# Autodesk Inventor assembly: black-suspension_MIR
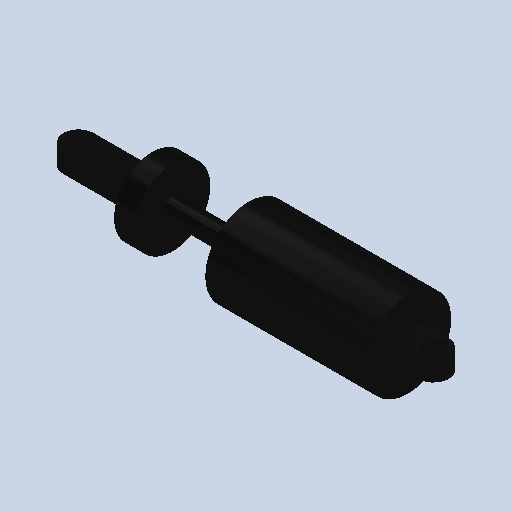
[picture p0: Inventor's stored thumbnail of the model, 512x512]
Saved by Autodesk Inventor 2025.1 (Build 291241000, 241)
## iProperties
Created: 2023-11-21
Part Number: black-suspension_MIR
Document SubType Name: Assembly
Designer: haruy
Author: haruy
## Documents named in this file (3)
- C:\Users\haruy\Documents\ロボコン\NHK2025\cad\000_parts\サスペンション\black-suspension_MIR.iam
- C:\Users\haruy\Documents\ロボコン\NHK2025\cad\000_parts\サスペンション\black-suspension-top_MIR.ipt
- C:\Users\haruy\Documents\ロボコン\NHK2025\cad\000_parts\サスペンション\black-suspension-under_MIR.ipt
## Components (2 placed, 2 different names)
1. black-suspension-top_MIR:1 — 角度:1, 円柱状:1
2. black-suspension-under_MIR:1 — 角度:1, 円柱状:1
## Relationships (2: Angle 1, CylindricalJoint 1)
- 角度:1 [Angle] (0 deg): black-suspension-top_MIR:1 ↔ black-suspension-under_MIR:1
- 円柱状:1 [CylindricalJoint]: black-suspension-top_MIR:1 ↔ black-suspension-under_MIR:1
